# Autodesk Inventor assembly: 3-finger_gripper_finger_C
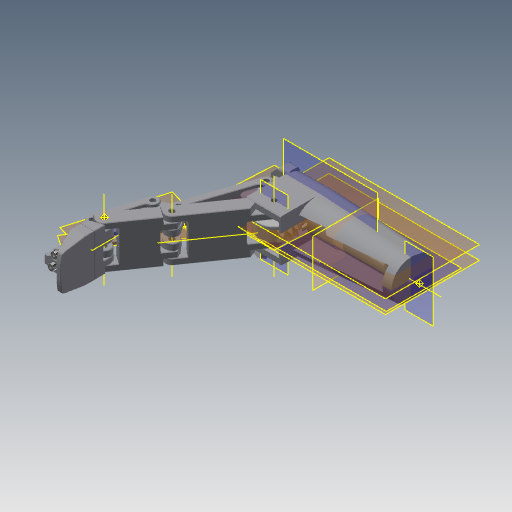
[picture p0: Inventor's stored thumbnail of the model, 512x512]
Saved by Autodesk Inventor 2018 (Build 220112000, 112)
## iProperties
Created: 2019-01-30
Part Number: 3-finger_gripper_finger_C
Document SubType Name: Assembly
Designer: Tsche
Author: Tsche
## Documents named in this file (20)
- C:\Users\Tsche\Documents\3d-printer\parts\grippers\Three_Finger_Gripper\BetaBots-Robot-Arm-Project-master\BetaBots-Robot-Arm-Project-master\ThreeFingerGripper\inventor\Gripper\cad_files\3-finger_gripper_finger_B.iam
- C:\Users\Tsche\Documents\3d-printer\parts\grippers\Three_Finger_Gripper\BetaBots-Robot-Arm-Project-master\BetaBots-Robot-Arm-Project-master\ThreeFingerGripper\inventor\Gripper\cad_files\finger_part_a.ipt
- C:\Users\Tsche\Documents\3d-printer\parts\grippers\Three_Finger_Gripper\BetaBots-Robot-Arm-Project-master\BetaBots-Robot-Arm-Project-master\ThreeFingerGripper\inventor\Gripper\cad_files\finger_part_b.ipt
- C:\Users\Tsche\Documents\3d-printer\parts\grippers\Three_Finger_Gripper\BetaBots-Robot-Arm-Project-master\BetaBots-Robot-Arm-Project-master\ThreeFingerGripper\inventor\Gripper\cad_files\finger_part_c.ipt
- C:\Users\Tsche\Documents\3d-printer\parts\grippers\Three_Finger_Gripper\BetaBots-Robot-Arm-Project-master\BetaBots-Robot-Arm-Project-master\ThreeFingerGripper\inventor\Gripper\cad_files\bar_bc.ipt
- C:\Users\Tsche\Documents\3d-printer\parts\grippers\Three_Finger_Gripper\BetaBots-Robot-Arm-Project-master\BetaBots-Robot-Arm-Project-master\ThreeFingerGripper\inventor\Gripper\cad_files\hinge_act_b.ipt
- C:\Users\Tsche\Documents\3d-printer\parts\grippers\Three_Finger_Gripper\BetaBots-Robot-Arm-Project-master\BetaBots-Robot-Arm-Project-master\ThreeFingerGripper\inventor\Gripper\cad_files\bar_act_ab.ipt
- C:\Users\Tsche\Documents\3d-printer\parts\grippers\Three_Finger_Gripper\BetaBots-Robot-Arm-Project-master\BetaBots-Robot-Arm-Project-master\ThreeFingerGripper\inventor\Gripper\cad_files\hinge_guid_b.ipt
- C:\Users\Tsche\Documents\3d-printer\parts\grippers\Three_Finger_Gripper\BetaBots-Robot-Arm-Project-master\BetaBots-Robot-Arm-Project-master\ThreeFingerGripper\inventor\Gripper\cad_files\bar_guid_ab.ipt
- C:\Users\Tsche\Documents\3d-printer\parts\grippers\Three_Finger_Gripper\BetaBots-Robot-Arm-Project-master\BetaBots-Robot-Arm-Project-master\ThreeFingerGripper\inventor\Gripper\cad_files\hinge_guid_a.ipt
- C:\Users\Tsche\Documents\3d-printer\parts\grippers\Three_Finger_Gripper\BetaBots-Robot-Arm-Project-master\BetaBots-Robot-Arm-Project-master\ThreeFingerGripper\inventor\Gripper\cad_files\hinge_guid_c.ipt
- C:\Users\Tsche\Documents\3d-printer\parts\grippers\Three_Finger_Gripper\BetaBots-Robot-Arm-Project-master\BetaBots-Robot-Arm-Project-master\ThreeFingerGripper\inventor\Gripper\cad_files\hinge_act_a2.ipt
- C:\Users\Tsche\Documents\3d-printer\parts\grippers\Three_Finger_Gripper\BetaBots-Robot-Arm-Project-master\BetaBots-Robot-Arm-Project-master\ThreeFingerGripper\inventor\Gripper\cad_files\worm.ipt
- C:\Users\Tsche\Documents\3d-printer\parts\grippers\Three_Finger_Gripper\BetaBots-Robot-Arm-Project-master\BetaBots-Robot-Arm-Project-master\ThreeFingerGripper\inventor\Gripper\cad_files\dc-motor_12V_60U-min.ipt
- C:\Users\Tsche\Documents\3d-printer\parts\grippers\Three_Finger_Gripper\BetaBots-Robot-Arm-Project-master\BetaBots-Robot-Arm-Project-master\ThreeFingerGripper\inventor\Gripper\cad_files\finger-main_B.ipt
- C:\Users\Tsche\Documents\3d-printer\parts\grippers\Three_Finger_Gripper\BetaBots-Robot-Arm-Project-master\BetaBots-Robot-Arm-Project-master\ThreeFingerGripper\inventor\Gripper\cad_files\tilt-gear_B.ipt
- C:\Users\Tsche\Documents\3d-printer\parts\grippers\Three_Finger_Gripper\BetaBots-Robot-Arm-Project-master\BetaBots-Robot-Arm-Project-master\ThreeFingerGripper\inventor\Gripper\cad_files\tilt-gear_B2.ipt
- C:\Users\Tsche\Documents\3d-printer\parts\grippers\Three_Finger_Gripper\BetaBots-Robot-Arm-Project-master\BetaBots-Robot-Arm-Project-master\ThreeFingerGripper\inventor\Gripper\cad_files\finger-tip_base.ipt
- C:\Users\Tsche\Documents\3d-printer\parts\grippers\Three_Finger_Gripper\BetaBots-Robot-Arm-Project-master\BetaBots-Robot-Arm-Project-master\ThreeFingerGripper\inventor\Gripper\cad_files\rotating_finger-tip\rotating_finger-tip_B.iam
- C:\Users\Tsche\Documents\3d-printer\parts\grippers\Three_Finger_Gripper\BetaBots-Robot-Arm-Project-master\BetaBots-Robot-Arm-Project-master\ThreeFingerGripper\inventor\Gripper\cad_files\Dimensions.xlsx
## Components (19 placed, 18 different names)
1. finger-main_B:1 — Cylindrical:20, Cylindrical:21, Mate:15, Angle:1, Mate:16, Mate:17, Mate:18, Mate:19, Mate:20, Angle:21, Cylindrical:16, Cylindrical:19
2. finger_part_a:1 — Cylindrical:1, Flush:1, Cylindrical:20, Mate:14
3. finger_part_b:1 — Cylindrical:1, Flush:1, Cylindrical:2, Mate:3, Cylindrical:4, Cylindrical:9
4. finger_part_c:1 — Cylindrical:2, Mate:3, Mate:4, Cylindrical:3, Cylindrical:14, Mate:21, Mate:22, Mate:23, Mate:24, Mate:25, Mate:26
5. bar_bc:1 — Mate:4, Cylindrical:3, Mate:5, Cylindrical:5, Mate:6, Flush:2
6. hinge_act_b:1 — Mate:5, Cylindrical:4, Cylindrical:5, Cylindrical:6
7. bar_act_ab:1 — Mate:6, Cylindrical:6, Mate:13, Cylindrical:18
8. bar_bc:2 — Flush:2, Mate:8, Cylindrical:10, Mate:11, Cylindrical:15
9. hinge_guid_b:1 — Mate:8, Cylindrical:9, Cylindrical:10, Mate:9, Cylindrical:11
10. bar_guid_ab:1 — Mate:9, Cylindrical:11, Flush:11, Cylindrical:17
11. hinge_guid_a:1 — Flush:11, Cylindrical:16, Cylindrical:17
12. hinge_guid_c:1 — Mate:11, Cylindrical:14, Cylindrical:15
13. Worm Gear:1 — Mate:13, Cylindrical:18, Cylindrical:19
14. Worm:2 — Cylindrical:21, Mate:14
15. dc-motor_12V_60U-min:1 — Mate:15, Angle:1, Mate:16
16. tilt-gear_B:1 — Mate:17, Angle:20, Mate:18
17. tilt-gear_B2:1 — Mate:19, Mate:20, Angle:21
18. finger-tip_base:1 — Mate:21, Mate:22, Mate:23
19. rotating_finger-tip_B:1 [sub-assembly] — Mate:24, Mate:25, Mate:26
## Relationships (45: Mate 21, CylindricalJoint 17, Flush 4, Angle 3)
- Cylindrical:1: finger_part_a:1 ↔ finger_part_b:1
- Flush:1: finger_part_a:1 ↔ finger_part_b:1
- Cylindrical:2: finger_part_b:1 ↔ finger_part_c:1
- Mate:3: finger_part_b:1 ↔ finger_part_c:1
- Mate:4: finger_part_c:1 ↔ bar_bc:1
- Cylindrical:3: finger_part_c:1 ↔ bar_bc:1
- Mate:5: bar_bc:1 ↔ hinge_act_b:1
- Cylindrical:4: finger_part_b:1 ↔ hinge_act_b:1
- Cylindrical:5: bar_bc:1 ↔ hinge_act_b:1
- Mate:6: bar_bc:1 ↔ bar_act_ab:1
- Cylindrical:6: hinge_act_b:1 ↔ bar_act_ab:1
- Flush:2 (8 mm): bar_bc:1 ↔ bar_bc:2
- Mate:8: bar_bc:2 ↔ hinge_guid_b:1
- Cylindrical:9: finger_part_b:1 ↔ hinge_guid_b:1
- Cylindrical:10: bar_bc:2 ↔ hinge_guid_b:1
- Mate:9: hinge_guid_b:1 ↔ bar_guid_ab:1
- Cylindrical:11: hinge_guid_b:1 ↔ bar_guid_ab:1
- Flush:11: bar_guid_ab:1 ↔ hinge_guid_a:1
- Mate:11: bar_bc:2 ↔ hinge_guid_c:1
- Cylindrical:14: finger_part_c:1 ↔ hinge_guid_c:1
- Cylindrical:15: bar_bc:2 ↔ hinge_guid_c:1
- Cylindrical:16: finger-main_B:1 ↔ hinge_guid_a:1
- Cylindrical:17: bar_guid_ab:1 ↔ hinge_guid_a:1
- Mate:13: bar_act_ab:1 ↔ Worm Gear:1
- Cylindrical:18: bar_act_ab:1 ↔ Worm Gear:1
- Cylindrical:19: finger-main_B:1 ↔ Worm Gear:1
- Cylindrical:20: finger-main_B:1 ↔ finger_part_a:1
- [Flush]: finger-main_B:1 ↔ finger_part_a:1
- Cylindrical:21: finger-main_B:1 ↔ Worm:2
- Mate:14: finger_part_a:1 ↔ Worm:2
- Mate:15: finger-main_B:1 ↔ dc-motor_12V_60U-min:1
- Angle:1 (0 deg): finger-main_B:1 ↔ dc-motor_12V_60U-min:1
- Mate:16: finger-main_B:1 ↔ dc-motor_12V_60U-min:1
- Mate:17: finger-main_B:1 ↔ tilt-gear_B:1
- Angle:20 (0 deg): tilt-gear_B:1
- Mate:18: finger-main_B:1 ↔ tilt-gear_B:1
- Mate:19: finger-main_B:1 ↔ tilt-gear_B2:1
- Mate:20: finger-main_B:1 ↔ tilt-gear_B2:1
- Angle:21 (0 deg): finger-main_B:1 ↔ tilt-gear_B2:1
- Mate:21: finger_part_c:1 ↔ finger-tip_base:1
- Mate:22: finger_part_c:1 ↔ finger-tip_base:1
- Mate:23: finger_part_c:1 ↔ finger-tip_base:1
- Mate:24: finger_part_c:1 ↔ rotating_finger-tip_B:1
- Mate:25: finger_part_c:1 ↔ rotating_finger-tip_B:1
- Mate:26: finger_part_c:1 ↔ rotating_finger-tip_B:1
## Named parameters: finger_width = 25 mm, finger_thickness = 8 mm, finger_part_A_length = 42.8625 mm, finger_part_B_length = 28.575 mm, finger_link_width = 3.5 mm, finger_link_clearence = 0.075 mm, tol = 0.0375 mm, link_tol = 0.254 mm, bore_press = 2.925 mm, bore_clearance = 3.025 mm, bar_diameter = 6.5 mm, bar_thickness = 4 mm, bar_width = 7 mm, hinge_dist_sym_plane = 4 mm, hinge_thickness = 3 mm, hinge_act_length_c = 7.62 mm, hinge_act_length_bc = 16.66875 mm, hinge_act_length_ab = 11.049 mm, hinge_act_length_a = 21.43125 mm, hinge_guid_length_c = 9.525 mm, hinge_guid_length_bc = 9.525 mm, hinge_guid_length_ab = 17.145 mm, hinge_guid_length_a = 17.145 mm, bar_length_bc = 28.575 mm, bar_act_length_ab = 40.48125 mm, bar_guid_length_ab = 43.275 mm, champfer = 0.3 mm, fillet = 0.4 mm, gear_diameter = 14 mm, dist_finger_BC = 56.5 mm, dist_hinge_points = 51.25 mm, hinge_point = 15 mm
